# Autodesk Inventor assembly: Rotation Resistor Assembly
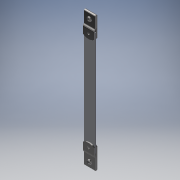
[picture p0: Inventor's stored thumbnail of the model, 180x180]
Saved by Autodesk Inventor 2018 (Build 220112000, 112)
## iProperties
Created: 2018-02-27
Part Number: Rotation Resistor Assembly
Document SubType Name: Assembly
Designer: 232963
Author: 232963
## Documents named in this file (3)
- P:\IED\SchoolCAD\ReverseEngineering\Rotation Resistor Assembly.iam
- P:\IED\SchoolCAD\ReverseEngineering\Rotation Resistor-01.ipt
- P:\IED\SchoolCAD\ReverseEngineering\yes.ipt
## Components (3 placed, 2 different names)
1. Rotation Resistor-01:1 — Insert:1, Flush:1, Insert:2, Flush:2
2. yes:1 — Insert:1, Flush:1
3. yes:2 — Insert:2, Flush:2
## Relationships (4: Insert 2, Flush 2)
- Insert:1: Rotation Resistor-01:1 ↔ yes:1
- Flush:1: Rotation Resistor-01:1 ↔ yes:1
- Insert:2: Rotation Resistor-01:1 ↔ yes:2
- Flush:2: Rotation Resistor-01:1 ↔ yes:2
